# Autodesk Inventor assembly: Base demo
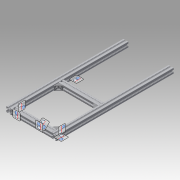
[picture p0: Inventor's stored thumbnail of the model, 180x180]
Saved by Autodesk Inventor 2016 (Build 200138000, 138)
## iProperties
Created: 2016-09-24
Part Number: Base demo
Document SubType Name: Assembly
Designer: Delta
Author: Delta
## Documents named in this file (4)
- C:\Robotics\2016-17_CAD\Base demo.iam
- C:\Users\Delta\Desktop\Bosch 20x20 17.5 in.ipt
- C:\Robotics\CAD\2015-16\COTSParts\Bosch Extrusion\Rexroth-Gusset with Fasteners (M4 x 8).ipt
- C:\Robotics\CAD\2015-16\COTSParts\Bosch Extrusion\Bosch 20x20.ipt
## Components (8 placed, 3 different names)
1. Rexroth-Gusset with Fasteners (M4 x 8):3 — Mate:4, Flush:2, Mate:5, Mate:6
2. Bosch 20x20:1 — Mate:2, Mate:3, Mate:6, Mate:7, Flush:3, Flush:4, Flush:9
3. Bosch 20x20 17.5 in:2 — Mate:4, Flush:2, Mate:5, Mate:7, Flush:3, Flush:7, Flush:11
4. Bosch 20x20 17.5 in:3 — Mate:1, Flush:1, Mate:3, Flush:4, Mate:13, Flush:8, Mate:14, Flush:9, Flush:10, Flush:12, Flush:13
5. Rexroth-Gusset with Fasteners (M4 x 8):1 — Mate:1, Flush:1, Mate:2
6. Bosch 20x20:2 — Mate:8, Flush:5, Mate:9, Flush:6, Mate:10, Mate:11, Mate:12, Flush:7, Flush:8, Mate:14, Flush:10, Flush:11, Flush:12, Flush:13
7. Rexroth-Gusset with Fasteners (M4 x 8):4 — Mate:8, Flush:5, Mate:10, Mate:11, Mate:13
8. Rexroth-Gusset with Fasteners (M4 x 8):5 — Mate:9, Flush:6, Mate:12
## Relationships (27: Mate 14, Flush 13)
- Mate:1: Bosch 20x20 17.5 in:3 ↔ Rexroth-Gusset with Fasteners (M4 x 8):1
- Flush:1 (20 mm): Bosch 20x20 17.5 in:3 ↔ Rexroth-Gusset with Fasteners (M4 x 8):1
- Mate:2: Bosch 20x20:1 ↔ Rexroth-Gusset with Fasteners (M4 x 8):1
- Mate:3: Bosch 20x20:1 ↔ Bosch 20x20 17.5 in:3
- Mate:4: Rexroth-Gusset with Fasteners (M4 x 8):3 ↔ Bosch 20x20 17.5 in:2
- Flush:2 (20 mm): Rexroth-Gusset with Fasteners (M4 x 8):3 ↔ Bosch 20x20 17.5 in:2
- Mate:5 (0.508 mm): Rexroth-Gusset with Fasteners (M4 x 8):3 ↔ Bosch 20x20 17.5 in:2
- Mate:6: Rexroth-Gusset with Fasteners (M4 x 8):3 ↔ Bosch 20x20:1
- Mate:7: Bosch 20x20:1 ↔ Bosch 20x20 17.5 in:2
- Flush:3: Bosch 20x20:1 ↔ Bosch 20x20 17.5 in:2
- Flush:4: Bosch 20x20:1 ↔ Bosch 20x20 17.5 in:3
- Mate:8: Bosch 20x20:2 ↔ Rexroth-Gusset with Fasteners (M4 x 8):4
- Flush:5: Bosch 20x20:2 ↔ Rexroth-Gusset with Fasteners (M4 x 8):4
- Mate:9: Bosch 20x20:2 ↔ Rexroth-Gusset with Fasteners (M4 x 8):5
- Flush:6: Bosch 20x20:2 ↔ Rexroth-Gusset with Fasteners (M4 x 8):5
- Mate:10 (6.5532 mm): Bosch 20x20:2 ↔ Rexroth-Gusset with Fasteners (M4 x 8):4
- Mate:11 (6.5532 mm): Bosch 20x20:2 ↔ Rexroth-Gusset with Fasteners (M4 x 8):4
- Mate:12 (0.1016 mm): Bosch 20x20:2 ↔ Rexroth-Gusset with Fasteners (M4 x 8):5
- Mate:13: Bosch 20x20 17.5 in:3 ↔ Rexroth-Gusset with Fasteners (M4 x 8):4
- Flush:7: Bosch 20x20 17.5 in:2 ↔ Bosch 20x20:2
- Flush:8: Bosch 20x20 17.5 in:3 ↔ Bosch 20x20:2
- Mate:14 (1.8034 mm): Bosch 20x20 17.5 in:3 ↔ Bosch 20x20:2
- Flush:9: Bosch 20x20:1 ↔ Bosch 20x20 17.5 in:3
- Flush:10: Bosch 20x20 17.5 in:3 ↔ Bosch 20x20:2
- Flush:11: Bosch 20x20 17.5 in:2 ↔ Bosch 20x20:2
- Flush:12: Bosch 20x20 17.5 in:3 ↔ Bosch 20x20:2
- Flush:13 (246.9388 mm): Bosch 20x20 17.5 in:3 ↔ Bosch 20x20:2
